# Autodesk Inventor assembly: Weapon (Weapon-Side Pulley)
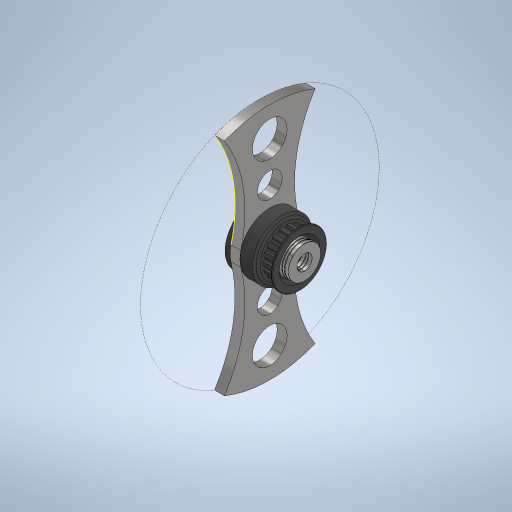
[picture p0: Inventor's stored thumbnail of the model, 512x512]
Saved by Autodesk Inventor 2023.2 (Build 272271000, 271)
## iProperties
Created: 2022-05-08
Part Number: Weapon (Weapon-Side Pulley)
Document SubType Name: Assembly
Designer: NCai2
Mass: 280.359 g
Surface Area: 311.324 cm^2
Volume: 49.83 cm^3
Density: 5.62632 g/cm^3
Author: NCai2
## Documents named in this file (6)
- E:\Documents\Inventor\0.3rd Lawette - V3.5\Vertical Weapon Assembly (3rd Law)\Weapon (Weapon-Side Pulley).iam
- E:\Documents\Inventor\0.3rd Lawette - V3.5\Vertical Weapon Assembly (3rd Law)\5905K132_Needle-Roller Bearing.ipt
- E:\Documents\Inventor\0.3rd Lawette - V3.5\Vertical Weapon Assembly (3rd Law)\Thrust Ball Bearing.ipt
- E:\Documents\Inventor\0.3rd Lawette - V3.5\Vertical Weapon Assembly (3rd Law)\Blade (Bar 2).ipt
- E:\Documents\Inventor\0.3rd Lawette - V3.5\Vertical Weapon Assembly (3rd Law)\Spacer 3-8x .125.ipt
- E:\Documents\Inventor\0.3rd Lawette - V3.5\Vertical Weapon Assembly (3rd Law)\XL Pulley 18T .25in Wd.ipt
## Components (7 placed, 5 different names)
1. 5905K132_Needle-Roller Bearing:5
2. 5905K132_Needle-Roller Bearing:6
3. Thrust Ball Bearing:5
4. Thrust Ball Bearing:6
5. Blade (Bar 2):2
6. Spacer 3-8x .125:2
7. XL Pulley 18T .25in Wd:2
## Relationships (15: Mate 15)
- [Mate]: 5905K132_Needle-Roller Bearing:6 ↔ Thrust Ball Bearing:5
- [Mate]: 5905K132_Needle-Roller Bearing:5 ↔ Thrust Ball Bearing:6
- [Mate]: 5905K132_Needle-Roller Bearing:6 ↔ Blade (Bar 2):2
- [Mate]: 5905K132_Needle-Roller Bearing:5 ↔ Thrust Ball Bearing:6
- [Mate]: 5905K132_Needle-Roller Bearing:5 ↔ 5905K132_Needle-Roller Bearing:6
- [Mate] (-38.1 mm): Thrust Ball Bearing:5 ↔ Thrust Ball Bearing:6
- [Mate]: 5905K132_Needle-Roller Bearing:6 ↔ Thrust Ball Bearing:5
- [Mate]: 5905K132_Needle-Roller Bearing:5 ↔ Spacer 3-8x .125:2
- [Mate]: Blade (Bar 2):2 ↔ Spacer 3-8x .125:2
- [Mate]: Blade (Bar 2):2 ↔ Spacer 3-8x .125:2
- [Mate]: Thrust Ball Bearing:6 ↔ Spacer 3-8x .125:2
- [Mate] (-34.925 mm): Thrust Ball Bearing:6 ↔ XL Pulley 18T .25in Wd:2
- [Mate]: Blade (Bar 2):2 ↔ XL Pulley 18T .25in Wd:2
- [Mate]: Blade (Bar 2):2 ↔ XL Pulley 18T .25in Wd:2
- [Mate]: 5905K132_Needle-Roller Bearing:5 ↔ 5905K132_Needle-Roller Bearing:6
